# Autodesk Inventor assembly: Assembly1
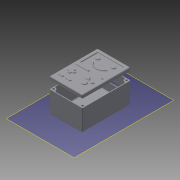
[picture p0: Inventor's stored thumbnail of the model, 180x180]
Saved by Autodesk Inventor 2015 (Build 190159000, 159)
## iProperties
Created: 2016-09-12
Part Number: Assembly1
Document SubType Name: Assembly
Designer: Administrator
Author: Administrator
## Documents named in this file (3)
- C:\Users\Administrator\Desktop\pieces\bemoo\Assembly1.iam
- C:\Users\Administrator\Desktop\pieces\bemoo\cuerpo.ipt
- C:\Users\Administrator\Desktop\pieces\bemoo\cara.ipt
## Components (2 placed, 2 different names)
1. cuerpo:1 — Flush:1, Flush:2, Mate:1
2. cara:1 — Flush:1, Flush:2, Mate:1
## Relationships (3: Flush 2, Mate 1)
- Flush:1: cuerpo:1 ↔ cara:1
- Flush:2: cuerpo:1 ↔ cara:1
- Mate:1 (20 mm): cuerpo:1 ↔ cara:1
